# Autodesk Inventor assembly: Engine
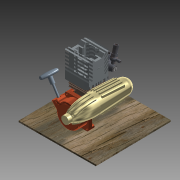
[picture p0: Inventor's stored thumbnail of the model, 180x180]
Saved by Autodesk Inventor 2015 (Build 190159000, 159)
## iProperties
Created: 2016-02-29
Part Number: Engine
Document SubType Name: Assembly
Designer: 672301
Author: 672301
## Documents named in this file (21)
- C:\Users\Owner\Desktop\Day1\Finalarm\Engine.iam
- C:\Users\Owner\Desktop\Day1\Finalarm\Engine Block.ipt
- C:\Users\Owner\Desktop\Day1\Finalarm\CrankShaft.ipt
- C:\Users\Owner\Desktop\Day1\Finalarm\Crankarm.ipt
- C:\Users\Owner\Desktop\Day1\Finalarm\Piston Shaft.ipt
- C:\Users\Owner\Desktop\Day1\Finalarm\Piston.ipt
- C:\Users\Owner\Desktop\Day1\Finalarm\pistopin.ipt
- C:\Users\Owner\Desktop\Day1\Finalarm\Face Plate.ipt
- C:\Users\Owner\Desktop\Day1\Finalarm\Starterhandle.ipt
- C:\Users\Owner\Desktop\Day1\Finalarm\Startercover.ipt
- C:\Users\Owner\Desktop\Day1\Finalarm\Carburetor Housing.ipt
- C:\Users\Owner\Desktop\Day1\Finalarm\Heatsink.ipt
- C:\Users\Owner\Desktop\Day1\Finalarm\Carburetor.ipt
- C:\Users\Owner\Desktop\Day1\Finalarm\Mixture  Control.ipt
- C:\Users\Owner\Desktop\Day1\Finalarm\Fuelintake.ipt
- C:\Users\Owner\Desktop\Day1\Finalarm\Fuel Adjuster.ipt
- C:\Users\Owner\Desktop\Day1\Finalarm\HexCap.ipt
- C:\Users\Owner\Desktop\Day1\Finalarm\MufflerMain.ipt
- C:\Users\Owner\Desktop\Day1\Finalarm\Mufflertip.ipt
- C:\Users\Owner\Desktop\Day1\Finalarm\Base.ipt
- C:\Users\Owner\Desktop\Day1\Finalarm\pulley shaft.ipt
## Components (20 placed, 20 different names)
1. Engine Block:1 — Insert:1, Insert:3, Insert:4, Mate:6, Insert:8, Insert:10, Insert:11, Angle:1, Mate:19
2. CrankShaft:1 — Insert:1, Insert:2, Rotation/Translation:1, Angle:7
3. Crankarm:1 — Insert:2, Mate:5, Insert:18
4. Piston Shaft:1 — Insert:3, Mate:4, Insert:14
5. Piston:1 — Mate:2, Mate:3, Mate:4
6. pistopin:1 — Mate:2, Mate:3, Mate:5
7. Face Plate:1 — Insert:4, Mate:6, Insert:5, Mate:7, Mate:18
8. Starterhandle:1 — Mate:8, Rotation/Translation:1, Mate:9
9. Startercover:1 — Insert:5, Mate:7, Mate:8, Mate:9
10. Heatsink:1 — Insert:14, Angle:1, Angle:4, Mate:20, Angle:5, Mate:21, Angle:6, Angle:7
11. Carburetor Housing:1 — Insert:8, Mate:10, Mate:11, Mate:12, Mate:13, Mate:14, Mate:15, Insert:16, Angle:4
12. Carburetor:1 — Mate:10, Mate:11, Mate:12, Mate:13, Angle:3
13. Mixture  Control:1 — Mate:14, Mate:15, Insert:9
14. Fuelintake:1 — Insert:16, Insert:17, Angle:2
15. Fuel Adjuster:1 — Insert:17, Angle:2, Angle:3
16. HexCap:1 — Insert:9
17. MufflerMain:1 — Insert:10, Insert:11, Insert:12, Mate:16, Mate:17, Insert:13
18. Mufflertip:1 — Insert:12, Mate:16, Mate:17, Insert:13
19. Base:1 — Mate:18
20. pulley shaft:1 — Insert:18, Mate:19
## Relationships (44: Mate 20, Insert 15, Angle 7, RelateRotateTranslate 1, Symmetry 1)
- Insert:1: Engine Block:1 ↔ CrankShaft:1
- Insert:2: CrankShaft:1 ↔ Crankarm:1
- Insert:3: Engine Block:1 ↔ Piston Shaft:1
- Mate:2: Piston:1 ↔ pistopin:1
- Mate:3: Piston:1 ↔ pistopin:1
- Mate:4: Piston Shaft:1 ↔ Piston:1
- Mate:5: Crankarm:1 ↔ pistopin:1
- Insert:4: Engine Block:1 ↔ Face Plate:1
- Mate:6: Engine Block:1 ↔ Face Plate:1
- Insert:5: Face Plate:1 ↔ Startercover:1
- Mate:7: Face Plate:1 ↔ Startercover:1
- Mate:8: Starterhandle:1 ↔ Startercover:1
- Rotation/Translation:1 [RelateRotateTranslate] (76.2 mm): CrankShaft:1 ↔ Starterhandle:1
- Mate:9: Starterhandle:1 ↔ Startercover:1
- Insert:8: Engine Block:1 ↔ Carburetor Housing:1
- Mate:10: Carburetor Housing:1 ↔ Carburetor:1
- Mate:11: Carburetor Housing:1 ↔ Carburetor:1
- Mate:12: Carburetor Housing:1 ↔ Carburetor:1
- Mate:13 (-1.27 mm): Carburetor Housing:1 ↔ Carburetor:1
- Mate:14: Carburetor Housing:1 ↔ Mixture  Control:1
- Mate:15: Carburetor Housing:1 ↔ Mixture  Control:1
- Insert:9: Mixture  Control:1 ↔ HexCap:1
- Insert:10: Engine Block:1 ↔ MufflerMain:1
- Insert:11: Engine Block:1 ↔ MufflerMain:1
- Insert:12: MufflerMain:1 ↔ Mufflertip:1
- Mate:16: MufflerMain:1 ↔ Mufflertip:1
- Mate:17: MufflerMain:1 ↔ Mufflertip:1
- Insert:13: MufflerMain:1 ↔ Mufflertip:1
- Insert:14: Piston Shaft:1 ↔ Heatsink:1
- Mate:18: Face Plate:1 ↔ Base:1
- Angle:1 (0 deg): Engine Block:1 ↔ Heatsink:1
- Insert:16: Carburetor Housing:1 ↔ Fuelintake:1
- Insert:17: Fuelintake:1 ↔ Fuel Adjuster:1
- Angle:2 (0 deg): Fuelintake:1 ↔ Fuel Adjuster:1
- Angle:3 (0 deg): Carburetor:1 ↔ Fuel Adjuster:1
- Angle:4 (0 deg): Heatsink:1 ↔ Carburetor Housing:1
- Insert:18: Crankarm:1 ↔ pulley shaft:1
- Mate:19: Engine Block:1 ↔ pulley shaft:1
- Mate:20: Heatsink:1
- Angle:5 (0 deg): Heatsink:1
- Mate:21: Heatsink:1
- Angle:6 (0 deg): Heatsink:1
- Symmetry:1
- Angle:7 (0 deg): CrankShaft:1 ↔ Heatsink:1
